# Autodesk Inventor assembly: Assembly1
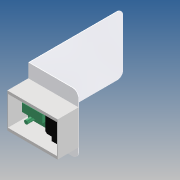
[picture p0: Inventor's stored thumbnail of the model, 180x180]
Saved by Autodesk Inventor 2020 (Build 240168000, 168)
## iProperties
Created: 2021-04-15
Part Number: Assembly1
Document SubType Name: Assembly
Designer: stephen
Author: stephen
## Documents named in this file (5)
- C:\Users\stephen\Documents\GitHub\Tumbler_Turner\3d_model\Assembly1.iam
- C:\Users\stephen\Documents\GitHub\Tumbler_Turner\3d_model\stepper_17HS4023.ipt
- C:\Users\stephen\Documents\GitHub\Tumbler_Turner\3d_model\pcb.ipt
- C:\Users\stephen\Documents\GitHub\Tumbler_Turner\3d_model\book_stand.ipt
- C:\Users\stephen\Documents\GitHub\Tumbler_Turner\3d_model\aluminium_project_box.ipt
## Components (4 placed, 4 different names)
1. stepper_17HS4023:1
2. pcb:1
3. book_stand:1 — Mate:1, Mate:2, Flush:1, Mate:6
4. aluminium_project_box:1 — Mate:6
## Relationships (4: Mate 3, Flush 1)
- Mate:1: book_stand:1
- Mate:2: book_stand:1
- Flush:1: book_stand:1
- Mate:6: book_stand:1 ↔ aluminium_project_box:1
